# Autodesk Inventor assembly: Maccaronikanone
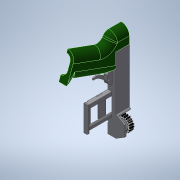
[picture p0: Inventor's stored thumbnail of the model, 180x180]
Saved by Autodesk Inventor 2021 (Build 250183000, 183)
## iProperties
Created: 2021-03-07
Part Number: Maccaronikanone
Document SubType Name: Assembly
Designer: Lukas
Author: Lukas
## Documents named in this file (15)
- \\192.168.1.200\Storragepool\Datastorrage\CAD\Inventor 2019\Maccaroni-Gun\Inventor files\Maccaronikanone.iam
- \\192.168.1.200\Storragepool\Datastorrage\CAD\Inventor 2019\Maccaroni-Gun\Inventor files\Abzug.ipt
- \\192.168.1.200\Storragepool\Datastorrage\CAD\Inventor 2019\Maccaroni-Gun\Inventor files\Maccaroni.ipt
- \\192.168.1.200\Storragepool\Datastorrage\CAD\Inventor 2019\Maccaroni-Gun\Inventor files\Motor_18mm.ipt
- \\192.168.1.200\Storragepool\Datastorrage\CAD\Inventor 2019\Maccaroni-Gun\Inventor files\Motor_holder.ipt
- \\192.168.1.200\Storragepool\Datastorrage\CAD\Inventor 2019\Maccaroni-Gun\Inventor files\Antriebsrad.ipt
- Z:\Datastorrage\CAD\Inventor 2019\Maccaroni-Gun\Inventor files\Abzugsgehäuse.ipt
- \\192.168.1.200\Storragepool\Datastorrage\CAD\Inventor 2019\Maccaroni-Gun\Inventor files\Magazin.ipt
- \\192.168.1.200\Storragepool\Datastorrage\CAD\Inventor 2019\Maccaroni-Gun\Inventor files\Magazin_Stössel.ipt
- \\192.168.1.200\Storragepool\Datastorrage\CAD\Inventor 2019\Maccaroni-Gun\Inventor files\Magazin_Boden.ipt
- \\192.168.1.200\Storragepool\Datastorrage\CAD\Inventor 2019\Maccaroni-Gun\Inventor files\Griff.ipt
- \\192.168.1.200\Storragepool\Datastorrage\CAD\Inventor 2019\Maccaroni-Gun\Inventor files\Hammer_Halter.ipt
- \\192.168.1.200\Storragepool\Datastorrage\CAD\Inventor 2019\Maccaroni-Gun\Inventor files\Abzug2.ipt
- \\192.168.1.200\Storragepool\Datastorrage\CAD\Inventor 2019\Maccaroni-Gun\Inventor files\Hammer2.ipt
- \\192.168.1.200\Storragepool\Datastorrage\CAD\Inventor 2019\Maccaroni-Gun\Inventor files\Abzughalter.ipt
## Components (16 placed, 14 different names)
1. Abzugsgehäuse:1 — Flush:1, Flush:2, Flush:3, Mate:61, Mate:62, Angle:1, Angle:2, Mate:69, Mate:70, Flush:6, Mate:72, Mate:74, Mate:75, Mate:76, Flush:9, Mate:77, Mate:78, Mate:82, Mate:83, Mate:84, Mate:86, Mate:88, Mate:89, Mate:90
2. Abzug:1 — Flush:9, Mate:77, Mate:78
3. Maccaroni:1 — Mate:63, Mate:70, Mate:71
4. Motor_holder:1 — Mate:55, Mate:56, Mate:57, Mate:58, Mate:59, Mate:60, Mate:61, Mate:62, Angle:1
5. Motor_18mm:1 — Mate:58, Mate:59, Mate:60, Insert:2, Mate:64
6. Motor_18mm:2 — Mate:55, Mate:56, Mate:57, Insert:1, Mate:65
7. Antriebsrad:1 — Insert:1, Mate:65
8. Antriebsrad:2 — Insert:2, Mate:64
9. Magazin:1 — Angle:2, Mate:68, Flush:5, Mate:69, Mate:71, Flush:6, Mate:72, Flush:7, Mate:73, Flush:8
10. Magazin_Stössel:1 — Mate:68, Flush:5
11. Magazin_Boden:1 — Flush:7, Mate:73, Flush:8
12. Griff:1 — Mate:74, Mate:75, Mate:76
13. Hammer_Halter:1 — Mate:82, Mate:83, Mate:84, Mate:87, Angle:3
14. Abzug2:1 — Mate:85, Mate:86, Tangent:1
15. Hammer2:1 — Mate:87, Angle:3, Tangent:1
16. Abzughalter:1 — Mate:88, Mate:85, Mate:89, Mate:90
## Relationships (45: Mate 31, Flush 8, Angle 3, Insert 2, Tangent 1)
- Flush:1: Abzugsgehäuse:1
- Flush:2: Abzugsgehäuse:1
- Flush:3: Abzugsgehäuse:1
- Mate:55: Motor_holder:1 ↔ Motor_18mm:2
- Mate:56: Motor_holder:1 ↔ Motor_18mm:2
- Mate:57: Motor_holder:1 ↔ Motor_18mm:2
- Mate:58: Motor_holder:1 ↔ Motor_18mm:1
- Mate:59: Motor_holder:1 ↔ Motor_18mm:1
- Mate:60: Motor_holder:1 ↔ Motor_18mm:1
- Mate:61: Abzugsgehäuse:1 ↔ Motor_holder:1
- Mate:62: Abzugsgehäuse:1 ↔ Motor_holder:1
- Angle:1 (0 deg): Abzugsgehäuse:1 ↔ Motor_holder:1
- Mate:63: Maccaroni:1
- Insert:1: Motor_18mm:2 ↔ Antriebsrad:1
- Insert:2: Motor_18mm:1 ↔ Antriebsrad:2
- Mate:64: Motor_18mm:1 ↔ Antriebsrad:2
- Mate:65: Motor_18mm:2 ↔ Antriebsrad:1
- Angle:2 (180 deg): Abzugsgehäuse:1 ↔ Magazin:1
- Mate:68: Magazin:1 ↔ Magazin_Stössel:1
- Flush:5: Magazin:1 ↔ Magazin_Stössel:1
- Mate:69 (0.1 mm): Abzugsgehäuse:1 ↔ Magazin:1
- Mate:70 (13 mm): Abzugsgehäuse:1 ↔ Maccaroni:1
- Mate:71: Maccaroni:1 ↔ Magazin:1
- Flush:6: Abzugsgehäuse:1 ↔ Magazin:1
- Mate:72: Abzugsgehäuse:1 ↔ Magazin:1
- Flush:7: Magazin:1 ↔ Magazin_Boden:1
- Mate:73: Magazin:1 ↔ Magazin_Boden:1
- Flush:8: Magazin:1 ↔ Magazin_Boden:1
- Mate:74: Abzugsgehäuse:1 ↔ Griff:1
- Mate:75: Abzugsgehäuse:1 ↔ Griff:1
- Mate:76: Abzugsgehäuse:1 ↔ Griff:1
- Flush:9: Abzugsgehäuse:1 ↔ Abzug:1
- Mate:77: Abzugsgehäuse:1 ↔ Abzug:1
- Mate:78: Abzugsgehäuse:1 ↔ Abzug:1
- Mate:82: Abzugsgehäuse:1 ↔ Hammer_Halter:1
- Mate:83: Abzugsgehäuse:1 ↔ Hammer_Halter:1
- Mate:84: Abzugsgehäuse:1 ↔ Hammer_Halter:1
- Mate:85: Abzug2:1 ↔ Abzughalter:1
- Mate:86 (0.1 mm): Abzugsgehäuse:1 ↔ Abzug2:1
- Mate:87: Hammer_Halter:1 ↔ Hammer2:1
- Angle:3 (0 deg): Hammer_Halter:1 ↔ Hammer2:1
- Tangent:1: Abzug2:1 ↔ Hammer2:1
- Mate:88: Abzugsgehäuse:1 ↔ Abzughalter:1
- Mate:89: Abzugsgehäuse:1 ↔ Abzughalter:1
- Mate:90: Abzugsgehäuse:1 ↔ Abzughalter:1
